# Autodesk Inventor assembly: Belt Tensioner 10mm
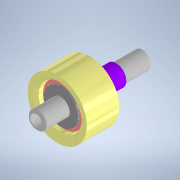
[picture p0: Inventor's stored thumbnail of the model, 180x180]
Saved by Autodesk Inventor 2022.2 (Build 262287000, 287)
## iProperties
Created: 2022-01-06
Part Number: Belt Tensioner 10mm
Document SubType Name: Assembly
Designer: Jochen
Author: Jochen
## Documents named in this file (7)
- D:\Projects\Lisbeth\CAD\Common\Belt Tensioner\BeltTensioner 10mm.iam
- D:\Projects\Lisbeth\CAD\Common\Belt Tensioner\BeltTensionerRoller 10mm.ipt
- D:\Projects\Lisbeth\CAD\Common\Bearing\bearing_7_3_3_sbn_683_2ZVA.ipt
- D:\Projects\Lisbeth\CAD\Common\Washer\Washer m2.5.ipt
- D:\Projects\Lisbeth\CAD\Common\Belt Tensioner\MotorBeltTensionerAxis.ipt
- D:\Projects\Lisbeth\CAD\Common\Belt Tensioner\OutputBeltTensionerSleeve 5mm.ipt
- D:\Projects\Lisbeth\CAD\Common\Belt Tensioner\MotorBeltTensionerGuide.ipt
## Components (6 placed, 6 different names)
1. Belt Tensioner 10mm:1
2. bearing_7_3_3_sbn_683_2ZVA:1 — Mate:9, Mate:20, Mate:24
3. Washer m2.5:1 — Mate:9, Mate:21
4. MotorBeltTensionerAxis:1 — Mate:20, Mate:21, Mate:23, Mate:25, Mate:26
5. OutputBeltTensionerSleeve 6mm:1 — Mate:23, Mate:24
6. MotorBeltTensionerGuide:1 — Mate:25, Mate:26
## Relationships (7: Mate 7)
- Mate:9: bearing_7_3_3_sbn_683_2ZVA:1 ↔ Washer m2.5:1
- Mate:20: bearing_7_3_3_sbn_683_2ZVA:1 ↔ MotorBeltTensionerAxis:1
- Mate:21 (4.15 mm): Washer m2.5:1 ↔ MotorBeltTensionerAxis:1
- Mate:23: MotorBeltTensionerAxis:1 ↔ OutputBeltTensionerSleeve 6mm:1
- Mate:24: bearing_7_3_3_sbn_683_2ZVA:1 ↔ OutputBeltTensionerSleeve 6mm:1
- Mate:25: MotorBeltTensionerAxis:1 ↔ MotorBeltTensionerGuide:1
- Mate:26: MotorBeltTensionerAxis:1 ↔ MotorBeltTensionerGuide:1
